# Autodesk Inventor assembly: kolko_do_wylania
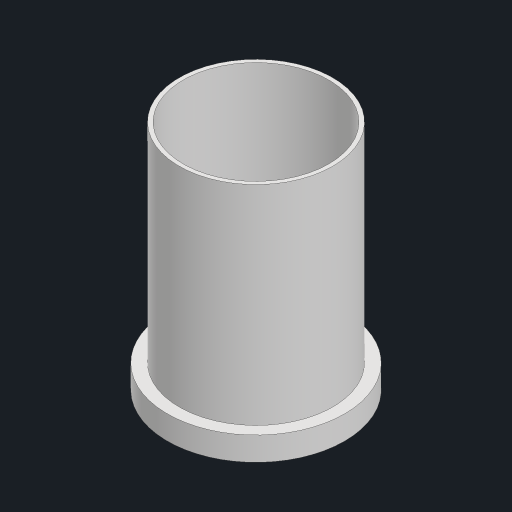
[picture p0: Inventor's stored thumbnail of the model, 512x512]
Saved by Autodesk Inventor 2023 (Build 270158000, 158)
## iProperties
Created: 2024-06-30
Part Number: kolko_do_wylania
Document SubType Name: Assembly
Designer: szymo
Author: szymo
## Documents named in this file (3)
- D:\roboilo\robots\codename wafel - australia\3d_parts\rev4\not_in_robot_parts\kolko_do_wylania_zlozenie.iam
- D:\roboilo\robots\codename wafel - australia\3d_parts\rev4\not_in_robot_parts\formaDoWylaniaSrodek.iam
- D:\roboilo\robots\codename wafel - australia\3d_parts\rev4\not_in_robot_parts\dol_do_wylania.ipt
## Components (2 placed, 2 different names)
1. formaDoWylaniaSrodek:1 [sub-assembly] — Flush:1
2. dol_do_wylania:1 — Flush:1
## Relationships (1: Flush 1)
- Flush:1: formaDoWylaniaSrodek:1 ↔ dol_do_wylania:1
